# Autodesk Inventor assembly: HeRoMini
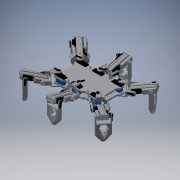
[picture p0: Inventor's stored thumbnail of the model, 180x180]
Saved by Autodesk Inventor 2017 (Build 210142000, 142)
## iProperties
Created: 2017-09-24
Part Number: HeRoMini
Document SubType Name: Assembly
Designer: Alexander Miller
Author: Alexander Miller
## Documents named in this file (3)
- X:\Alex\Documents\Git\HeRo-Mini\Hardware\HeRoMini.iam
- X:\Alex\Documents\Git\HeRo-Mini\Hardware\BODY.iam
- X:\Alex\Documents\Git\HeRo-Mini\Hardware\LEG.iam
## Components (7 placed, 2 different names)
1. BODY:1 [sub-assembly] — Rigid:2, Rigid:3, Rigid:4, Rigid:5, Rigid:6, Rigid:7
2. LEG:1 [sub-assembly] — Rigid:7
3. LEG:2 [sub-assembly] — Rigid:2
4. LEG:3 [sub-assembly] — Rigid:3
5. LEG:4 [sub-assembly] — Rigid:4
6. LEG:5 [sub-assembly] — Rigid:5
7. LEG:6 [sub-assembly] — Rigid:6
## Relationships (6: WeldJoint 6)
- Rigid:2 [WeldJoint]: BODY:1 ↔ LEG:2
- Rigid:3 [WeldJoint]: BODY:1 ↔ LEG:3
- Rigid:4 [WeldJoint]: BODY:1 ↔ LEG:4
- Rigid:5 [WeldJoint]: BODY:1 ↔ LEG:5
- Rigid:6 [WeldJoint]: BODY:1 ↔ LEG:6
- Rigid:7 [WeldJoint]: BODY:1 ↔ LEG:1
